# Autodesk Inventor assembly: CLB_075_ScissorLowBarAssembly
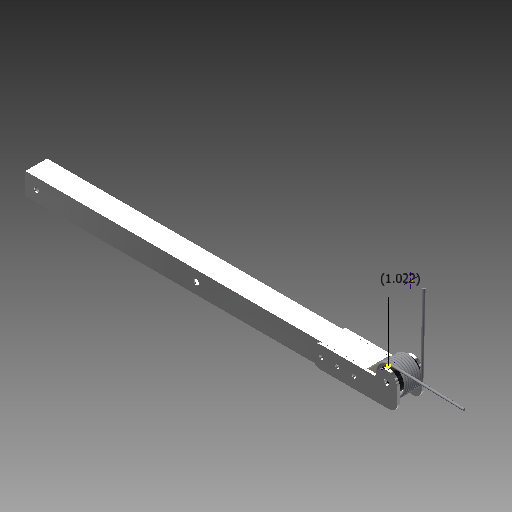
[picture p0: Inventor's stored thumbnail of the model, 512x512]
Saved by Autodesk Inventor 2018 (Build 220112000, 112)
## iProperties
Created: 2020-02-13
Part Number: CLB_075_ScissorLowBarAssembly
Document SubType Name: Assembly
Designer: Cooper
Author: Cooper
## Documents named in this file (8)
- C:\Users\Cooper\Documents\GrabCAD\Infinite Recharge 2020\Build season\CLB_075_ScissorLowBarAssembly.iam
- C:\Users\Cooper\Documents\GrabCAD\Infinite Recharge 2020\Build season\CLB_027_LifterBracket.ipt
- C:\Users\Cooper\Documents\GrabCAD\Infinite Recharge 2020\Build season\CLB_052_ScissorLiftPlug.ipt
- C:\Users\Cooper\Documents\GrabCAD\Infinite Recharge 2020\Build season\CLB_042_BottomBarFourPartScissors.ipt
- C:\Users\Cooper\Documents\GrabCAD\Infinite Recharge 2020\Build season\CLB_078_ScissorBottomBarPlug.ipt
- C:\Users\Cooper\Documents\GrabCAD\Infinite Recharge 2020\Build season\CLB_045_TorsionSpring_MM_9271K129.ipt
- C:\Users\Cooper\Documents\GrabCAD\Infinite Recharge 2020\Build season\CLB_047_SpringSpacer.ipt
- CLB_027_LifterBracket.ipt
## Components (7 placed, 6 different names)
1. CLB_042_BottomBarFourPartScissors:1 — Mate:3, Flush:2, Mate:4, Flush:3, Flush:4, Angle:1, Mate:45, Mate:46, Flush:50, Flush:51, Angle:2, Flush:53
2. CLB_027_LifterBracket:1 — Mate:3, Flush:2, Angle:1, Flush:51, Flush:52, Flush:54
3. CLB_027_LifterBracket:4 — Mate:4, Flush:3, Flush:4, Flush:52, Insert:1
4. CLB_052_ScissorLiftPlug:6 — Mate:45, Mate:46, Flush:50
5. CLB_078_ScissorBottomBarPlug:1 — Angle:2, Flush:53
6. CLB_045_TorsionSpring_MM_9271K129:1 — Mate:47, Flush:54
7. CLB_047_SpringSpacer:1 — Insert:1, Mate:47
## Relationships (16: Flush 8, Mate 5, Angle 2, Insert 1)
- Mate:3: CLB_042_BottomBarFourPartScissors:1 ↔ CLB_027_LifterBracket:1
- Flush:2 (-38.1 mm): CLB_042_BottomBarFourPartScissors:1 ↔ CLB_027_LifterBracket:1
- Mate:4: CLB_042_BottomBarFourPartScissors:1 ↔ CLB_027_LifterBracket:4
- Flush:3: CLB_042_BottomBarFourPartScissors:1 ↔ CLB_027_LifterBracket:4
- Flush:4 (-38.1 mm): CLB_042_BottomBarFourPartScissors:1 ↔ CLB_027_LifterBracket:4
- Angle:1 (0 deg): CLB_042_BottomBarFourPartScissors:1 ↔ CLB_027_LifterBracket:1
- Mate:45: CLB_042_BottomBarFourPartScissors:1 ↔ CLB_052_ScissorLiftPlug:6
- Mate:46: CLB_042_BottomBarFourPartScissors:1 ↔ CLB_052_ScissorLiftPlug:6
- Flush:50: CLB_042_BottomBarFourPartScissors:1 ↔ CLB_052_ScissorLiftPlug:6
- Flush:51: CLB_042_BottomBarFourPartScissors:1 ↔ CLB_027_LifterBracket:1
- Flush:52: CLB_027_LifterBracket:1 ↔ CLB_027_LifterBracket:4
- Angle:2 (0 deg): CLB_042_BottomBarFourPartScissors:1 ↔ CLB_078_ScissorBottomBarPlug:1
- Flush:53: CLB_042_BottomBarFourPartScissors:1 ↔ CLB_078_ScissorBottomBarPlug:1
- Insert:1: CLB_027_LifterBracket:4 ↔ CLB_047_SpringSpacer:1
- Mate:47: CLB_045_TorsionSpring_MM_9271K129:1 ↔ CLB_047_SpringSpacer:1
- Flush:54 (-2.54 mm): CLB_027_LifterBracket:1 ↔ CLB_045_TorsionSpring_MM_9271K129:1
